# Autodesk Inventor assembly: Złożenie ramienia robota
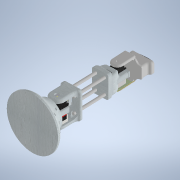
[picture p0: Inventor's stored thumbnail of the model, 180x180]
Saved by Autodesk Inventor 2021 (Build 250183000, 183)
## iProperties
Created: 2021-11-03
Part Number: Złożenie ramienia robota
Document SubType Name: Assembly
Designer: Łukasz
Author: Łukasz
## Documents named in this file (17)
- E:\GITHUB_Czołg\Szybki-Czolg-antyRadziecki\Ramie robota\Ramie robota\Złożenie ramienia robota.iam
- E:\GITHUB_Czołg\Szybki-Czolg-antyRadziecki\Ramie robota\Ramie robota\Podstawa 01-1.ipt
- E:\GITHUB_Czołg\Szybki-Czolg-antyRadziecki\Ramie robota\Ramie robota\Podstawa 01-2.ipt
- E:\GITHUB_Czołg\Szybki-Czolg-antyRadziecki\Ramie robota\Ramie robota\serwo 30x70.ipt
- E:\GITHUB_Czołg\Szybki-Czolg-antyRadziecki\Ramie robota\Ramie robota\mocowanie lozyska 10-1.ipt
- C:\Users\Łukasz\Documents\Inventor\Content Center Files\R2021\en-US\BS 292 (I)\BS 292 Part 1 - 608 - 8 x 22 x 7.ipt
- E:\GITHUB_Czołg\Szybki-Czolg-antyRadziecki\Ramie robota\Ramie robota\orczyk serwa okrągły 02-1.ipt
- E:\GITHUB_Czołg\Szybki-Czolg-antyRadziecki\Ramie robota\Ramie robota\ramie 03-1.ipt
- C:\Users\Łukasz\Documents\Inventor\Content Center Files\R2021\en-US\AS 1427(02)\AS 1427 - M8 x 16(2).ipt
- E:\GITHUB_Czołg\Szybki-Czolg-antyRadziecki\Ramie robota\Ramie robota\pręt 04-1.ipt
- E:\GITHUB_Czołg\Szybki-Czolg-antyRadziecki\Ramie robota\Ramie robota\podstawa 01-3.ipt
- E:\GITHUB_Czołg\Szybki-Czolg-antyRadziecki\Ramie robota\Ramie robota\servo 20x40.ipt
- E:\GITHUB_Czołg\Szybki-Czolg-antyRadziecki\Ramie robota\Ramie robota\ramie 03-2.ipt
- E:\GITHUB_Czołg\Szybki-Czolg-antyRadziecki\Ramie robota\Ramie robota\ramie 03-3.ipt
- E:\GITHUB_Czołg\Szybki-Czolg-antyRadziecki\Ramie robota\Ramie robota\mocowanie lozyska 10-2.ipt
- E:\GITHUB_Czołg\Szybki-Czolg-antyRadziecki\Ramie robota\Ramie robota\orczyk serwa okrągły 02-2.ipt
- E:\GITHUB_Czołg\Szybki-Czolg-antyRadziecki\Ramie robota\Ramie robota\ramie 03-4.ipt
## Components (21 placed, 16 different names)
1. Podstawa 01-1:1 — Mate:1, Mate:2, Mate:3
2. Podstawa 01-2:1 — Mate:4, Mate:5, Mate:6
3. serwo 30x70:1 — Mate:1, Mate:2, Mate:3, Mate:4, Mate:5, Mate:6, Mate:7, Flush:2, Rotational:2, Mate:8, Mate:9, Mate:10, Mate:11
4. mocowanie lozyska 10-1:1 — Mate:7, Flush:2, Rotational:1, Mate:8
5. BS 292: Part 1 (I) (Metric) 608 - 8 x 22 x 7:1 — Rotational:1
6. orczyk serwa okrągły 02-1:1 — Rotational:2, Rotational:9
7. ramie 03-1:1 — Rigid:1, Rigid:2, Rigid:3, Rigid:4, Rotational:9, Rotational:10
8. AS 1427 - Metric M8 x 16:1 — Rotational:10
9. pręt 04-1:1 — Rigid:1, Rotational:11
10. pręt 04-1:2 — Rigid:2, Rotational:12
11. pręt 04-1:3 — Rigid:3
12. pręt 04-1:4 — Rigid:4
13. podstawa 01-3:1 — Mate:9, Mate:10, Mate:11
14. servo 20x40:1 — Mate:12, Mate:13, Mate:14, Mate:15, Mate:16, Mate:17, Mate:18, Rotational:7
15. ramie 03-2:1 — Mate:12, Mate:13, Mate:14, Flush:3, Flush:4, Rotational:11, Rotational:12
16. ramie 03-3:1 — Mate:15, Flush:3, Flush:4
17. mocowanie lozyska 10-2:1 — Mate:16, Mate:17, Mate:18, Rotational:8
18. orczyk serwa okrągły 02-2:1 — Rotational:7, Rotational:13
19. BS 292: Part 1 (I) (Metric) 608 - 8 x 22 x 7:2 — Rotational:8
20. ramie 03-4:1 — Mate:19, Mate:20, Mate:21, Rotational:13
21. servo 20x40:2 — Mate:19, Mate:20, Mate:21
## Relationships (37: Mate 21, RevoluteJoint 9, WeldJoint 4, Flush 3)
- Mate:1: Podstawa 01-1:1 ↔ serwo 30x70:1
- Mate:2: Podstawa 01-1:1 ↔ serwo 30x70:1
- Mate:3: Podstawa 01-1:1 ↔ serwo 30x70:1
- Mate:4: Podstawa 01-2:1 ↔ serwo 30x70:1
- Mate:5: Podstawa 01-2:1 ↔ serwo 30x70:1
- Mate:6: Podstawa 01-2:1 ↔ serwo 30x70:1
- Mate:7: serwo 30x70:1 ↔ mocowanie lozyska 10-1:1
- Flush:2: serwo 30x70:1 ↔ mocowanie lozyska 10-1:1
- Rotational:1 [RevoluteJoint]: mocowanie lozyska 10-1:1 ↔ BS 292: Part 1 (I) (Metric) 608 - 8 x 22 x 7:1
- Rotational:2 [RevoluteJoint]: serwo 30x70:1 ↔ orczyk serwa okrągły 02-1:1
- Mate:8: serwo 30x70:1 ↔ mocowanie lozyska 10-1:1
- Rigid:1 [WeldJoint] (5 mm): ramie 03-1:1 ↔ pręt 04-1:1
- Rigid:2 [WeldJoint] (5 mm): ramie 03-1:1 ↔ pręt 04-1:2
- Rigid:3 [WeldJoint] (5 mm): ramie 03-1:1 ↔ pręt 04-1:3
- Rigid:4 [WeldJoint] (5 mm): ramie 03-1:1 ↔ pręt 04-1:4
- Mate:9: serwo 30x70:1 ↔ podstawa 01-3:1
- Mate:10: serwo 30x70:1 ↔ podstawa 01-3:1
- Mate:11: serwo 30x70:1 ↔ podstawa 01-3:1
- Mate:12: servo 20x40:1 ↔ ramie 03-2:1
- Mate:13: servo 20x40:1 ↔ ramie 03-2:1
- Mate:14: servo 20x40:1 ↔ ramie 03-2:1
- Mate:15: servo 20x40:1 ↔ ramie 03-3:1
- Flush:3: ramie 03-2:1 ↔ ramie 03-3:1
- Flush:4: ramie 03-2:1 ↔ ramie 03-3:1
- Mate:16: servo 20x40:1 ↔ mocowanie lozyska 10-2:1
- Mate:17: servo 20x40:1 ↔ mocowanie lozyska 10-2:1
- Mate:18: servo 20x40:1 ↔ mocowanie lozyska 10-2:1
- Rotational:7 [RevoluteJoint]: servo 20x40:1 ↔ orczyk serwa okrągły 02-2:1
- Rotational:8 [RevoluteJoint]: mocowanie lozyska 10-2:1 ↔ BS 292: Part 1 (I) (Metric) 608 - 8 x 22 x 7:2
- Rotational:9 [RevoluteJoint]: orczyk serwa okrągły 02-1:1 ↔ ramie 03-1:1
- Rotational:10 [RevoluteJoint]: ramie 03-1:1 ↔ AS 1427 - Metric M8 x 16:1
- Rotational:11 [RevoluteJoint]: pręt 04-1:1 ↔ ramie 03-2:1
- Rotational:12 [RevoluteJoint]: pręt 04-1:2 ↔ ramie 03-2:1
- Mate:19: ramie 03-4:1 ↔ servo 20x40:2
- Mate:20: ramie 03-4:1 ↔ servo 20x40:2
- Mate:21: ramie 03-4:1 ↔ servo 20x40:2
- Rotational:13 [RevoluteJoint]: orczyk serwa okrągły 02-2:1 ↔ ramie 03-4:1
